# Autodesk Inventor assembly: adjustable_connector
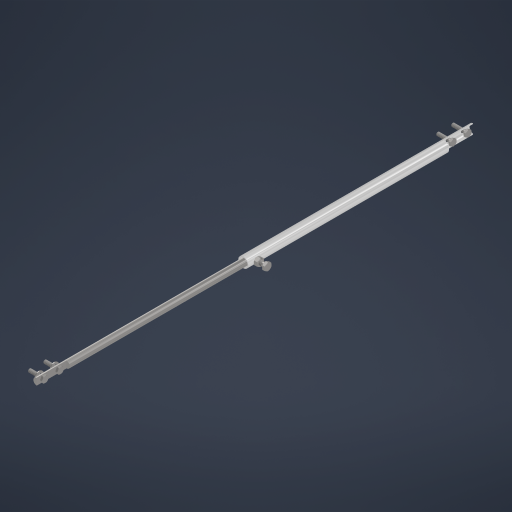
[picture p0: Inventor's stored thumbnail of the model, 512x512]
Saved by Autodesk Inventor 2023 (Build 270158000, 158)
## iProperties
Created: 2022-04-27
Part Number: adjustable_connector
Document SubType Name: Assembly
Designer: Norbert Ligas
connector_min_length: 306,147 mm
connector_max_length: 522,293 mm
Author: Norbert Ligas
## Documents named in this file (7)
- C:\Users\norbe\Repozytoria\NormalMapScanner\stand_construction\parts\adjustable_connector.iam
- C:\Users\norbe\Repozytoria\NormalMapScanner\stand_construction\parts\bar_connector.ipt
- C:\Users\norbe\Repozytoria\NormalMapScanner\stand_construction\parts\pipe_connector.ipt
- C:\Users\norbe\OneDrive\Dokumenty\Inventor\Content Center Files\R2023\en-US\ISO 4032(2)\ISO 4032 - M5 - ISO.ipt
- C:\Users\norbe\OneDrive\Dokumenty\Inventor\Content Center Files\R2023\en-US\ISO 4017(1)\ISO 4017 - M5 x 16 - ISO.ipt
- C:\Users\norbe\OneDrive\Dokumenty\Inventor\Content Center Files\R2023\en-US\ISO 4017(1)\ISO 4017 - M4 x 16 - ISO.ipt
- C:\Users\norbe\OneDrive\Dokumenty\Inventor\Content Center Files\R2023\en-US\ISO 7089\ISO 7089 - 5 - 140 HV(1).ipt
## Components (10 placed, 6 different names)
1. bar_connector:1 — Cylindrical:1, Flush:1, Insert:2, Insert:3, Tangent:2
2. pipe_connector:1 — Mate:4, Mate:5, Cylindrical:1, Flush:1, Mate:6, Tangent:1, Angle:1, Mate:7, Mate:8, Mate:9, Mate:10
3. ISO 4032 M5:1 — Mate:6, Tangent:1, Angle:1, Insert:1
4. ISO 4017 M5 x 16:1 — Insert:1
5. ISO 4017 M4 x 16:1 — Insert:3, Mate:12
6. ISO 4017 M4 x 16:2 — Insert:2, Mate:11
7. ISO 4017 M4 x 16:3 — Mate:7, Mate:8
8. ISO 4017 M4 x 16:4 — Mate:9, Mate:10
9. ISO 7089 5:1 — Mate:11, Flush:2
10. ISO 7089 5:2 — Mate:12, Flush:3
## Relationships (20: Mate 9, Flush 3, Insert 3, Tangent 2, Angle 2, CylindricalJoint 1)
- Mate:4: pipe_connector:1
- Mate:5: pipe_connector:1
- Cylindrical:1: bar_connector:1 ↔ pipe_connector:1
- Flush:1: bar_connector:1 ↔ pipe_connector:1
- Mate:6: pipe_connector:1 ↔ ISO 4032 M5:1
- Tangent:1: pipe_connector:1 ↔ ISO 4032 M5:1
- Angle:1 (90 deg): pipe_connector:1 ↔ ISO 4032 M5:1
- Insert:1 (5 mm): ISO 4032 M5:1 ↔ ISO 4017 M5 x 16:1
- Insert:2: bar_connector:1 ↔ ISO 4017 M4 x 16:2
- Insert:3: bar_connector:1 ↔ ISO 4017 M4 x 16:1
- Mate:7: pipe_connector:1 ↔ ISO 4017 M4 x 16:3
- Mate:8: pipe_connector:1 ↔ ISO 4017 M4 x 16:3
- Mate:9: pipe_connector:1 ↔ ISO 4017 M4 x 16:4
- Mate:10: pipe_connector:1 ↔ ISO 4017 M4 x 16:4
- Mate:11: ISO 4017 M4 x 16:2 ↔ ISO 7089 5:1
- Mate:12: ISO 4017 M4 x 16:1 ↔ ISO 7089 5:2
- Angle:2 (0 deg)
- Tangent:2: bar_connector:1
- Flush:2: ISO 7089 5:1
- Flush:3: ISO 7089 5:2
## Named parameters: min_extrusion = 35 mm, max_extrusion = 251.14675 mm, connector_min_length = 306.14675 mm, connector_max_length = 522.29349 mm, bar_length = 271.14675 mm, pipe_length = 271.14675 mm, bar_connection = 35 mm, pipe_connection = 35 mm, bar_pipe_connection_length = 20 mm
